# Autodesk Inventor assembly: marco
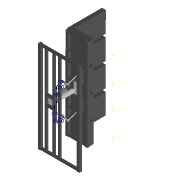
[picture p0: Inventor's stored thumbnail of the model, 180x180]
Saved by Autodesk Inventor 2021 (Build 250183000, 183)
## iProperties
Created: 2021-04-11
Part Number: marco
Document SubType Name: Assembly
Designer: equip
Mass: 525959 g
Surface Area: 133006 cm^2
Volume: 315655 cm^3
Density: 1.66625 g/cm^3
_SolveAssemblyDoc: Frame Generator Solve Assembly
_Version: 25.0.0
Author: equip
## Documents named in this file (13)
- C:\Users\Santiago Suárez\Documents\GitHub\Dis.-Mecatronico-E6\inventor proyecto\marco.iam
- C:\Users\Santiago Suárez\Documents\GitHub\Dis.-Mecatronico-E6\inventor proyecto\placa centro.ipt
- C:\Users\Santiago Suárez\Documents\GitHub\Dis.-Mecatronico-E6\inventor proyecto\Silla del marco.ipt
- C:\Users\Santiago Suárez\Documents\GitHub\Dis.-Mecatronico-E6\inventor proyecto\cilindro\cilindro.iam
- C:\Users\Santiago Suárez\Documents\GitHub\Dis.-Mecatronico-E6\inventor proyecto\marco inferior.ipt
- C:\Users\Santiago Suárez\Documents\GitHub\Dis.-Mecatronico-E6\inventor proyecto\marco\Frame\Marco Inferior.iam
- C:\Users\Santiago Suárez\Documents\GitHub\Dis.-Mecatronico-E6\inventor proyecto\MarcoSuperior.iam
- C:\Users\Santiago Suárez\Documents\GitHub\Dis.-Mecatronico-E6\inventor proyecto\Motor1.ipt
- C:\Users\Santiago Suárez\Documents\GitHub\Dis.-Mecatronico-E6\inventor proyecto\PlacaInferior.ipt
- C:\Users\Santiago Suárez\Documents\GitHub\Dis.-Mecatronico-E6\inventor proyecto\Eje.ipt
- C:\Users\Santiago Suárez\Documents\GitHub\Dis.-Mecatronico-E6\inventor proyecto\manivela.ipt
- C:\Users\Santiago Suárez\Documents\GitHub\Dis.-Mecatronico-E6\inventor proyecto\Biela.iam
- C:\Users\Santiago Suárez\Documents\GitHub\Dis.-Mecatronico-E6\inventor proyecto\UnionMarco.ipt
## Components (21 placed, 12 different names)
1. placa centro:1 — Rigid:3, Rigid:8
2. marco inferior:1
3. Marco Inferior:1 [sub-assembly] — Mate:23, Mate:24
4. MarcoSuperior:1 [sub-assembly] — Rigid:3, Mate:21, Mate:22, Mate:28, Mate:29, Mate:31, Mate:32, Mate:33, Mate:34
5. Motor1:1 — Rigid:5, Rotational:1, Rotational:2
6. PlacaInferior:1 — Mate:23, Mate:24, Mate:25, Mate:26, Mate:27, Rigid:5
7. cilindro:1 [sub-assembly] — Mate:25, Mate:26, Mate:27, Rigid:8
8. Eje:1 — Rotational:1, Rigid:9
9. Eje:2 — Rotational:2, Rigid:10
10. manivela:1 — Rigid:10, Rigid:11
11. manivela:2 — Rigid:9, Rigid:12
12. Biela:1 [sub-assembly] — Rigid:11, Rigid:18
13. Biela:2 [sub-assembly] — Rigid:12, Rigid:17
14. UnionMarco:1 — Rigid:13, Mate:28, Mate:29, Mate:34
15. UnionMarco:2 — Rigid:15, Mate:31, Mate:32, Mate:33
16. Eje:3 — Rigid:13, Rigid:17
17. Eje:4 — Rigid:15, Rigid:18
18. Silla del marco:1 — Mate:21, Mate:22
19. Silla del marco:2
20. Silla del marco:3
21. Silla del marco:4
## Component patterns: (4 elements, first: Silla del marco:1)
## Relationships (26: Mate 13, WeldJoint 11, RevoluteJoint 2)
- Rigid:3 [WeldJoint]: placa centro:1 ↔ MarcoSuperior:1
- Mate:21 (-10 mm): MarcoSuperior:1 ↔ Silla del marco:1
- Mate:22: MarcoSuperior:1 ↔ Silla del marco:1
- Mate:23: Marco Inferior:1 ↔ PlacaInferior:1
- Mate:24: Marco Inferior:1 ↔ PlacaInferior:1
- Mate:25: PlacaInferior:1 ↔ cilindro:1
- Mate:26 (88.5 mm): PlacaInferior:1 ↔ cilindro:1
- Mate:27 (-100 mm): PlacaInferior:1 ↔ cilindro:1
- Rigid:5 [WeldJoint]: Motor1:1 ↔ PlacaInferior:1
- Rotational:1 [RevoluteJoint]: Motor1:1 ↔ Eje:1
- Rotational:2 [RevoluteJoint]: Motor1:1 ↔ Eje:2
- Rigid:8 [WeldJoint]: placa centro:1 ↔ cilindro:1
- Rigid:9 [WeldJoint]: Eje:1 ↔ manivela:2
- Rigid:10 [WeldJoint]: Eje:2 ↔ manivela:1
- Rigid:11 [WeldJoint] (3 mm): manivela:1 ↔ Biela:1
- Rigid:12 [WeldJoint] (-3 mm): manivela:2 ↔ Biela:2
- Rigid:13 [WeldJoint] (-3 mm): UnionMarco:1 ↔ Eje:3
- Rigid:15 [WeldJoint] (3 mm): UnionMarco:2 ↔ Eje:4
- Rigid:17 [WeldJoint]: Biela:2 ↔ Eje:3
- Rigid:18 [WeldJoint]: Biela:1 ↔ Eje:4
- Mate:28: MarcoSuperior:1 ↔ UnionMarco:1
- Mate:29 (250 mm): MarcoSuperior:1 ↔ UnionMarco:1
- Mate:31: MarcoSuperior:1 ↔ UnionMarco:2
- Mate:32 (250 mm): MarcoSuperior:1 ↔ UnionMarco:2
- Mate:33 (8.5 mm): MarcoSuperior:1 ↔ UnionMarco:2
- Mate:34 (8.5 mm): MarcoSuperior:1 ↔ UnionMarco:1
## Named parameters: sa_0 = 470880, sa_1 = 470880, sa_2 = 470880, sa_3 = 470880, sa_4 = 1000, sa_5 = 1e+06, sa_6 = 1e+06
note: some values were not read from the file. Shown as the stored number, unit unknown: "sa_0", "sa_1", "sa_2", "sa_3", "sa_4", "sa_5", "sa_6".
